# Autodesk Inventor assembly: Ensamblaje4
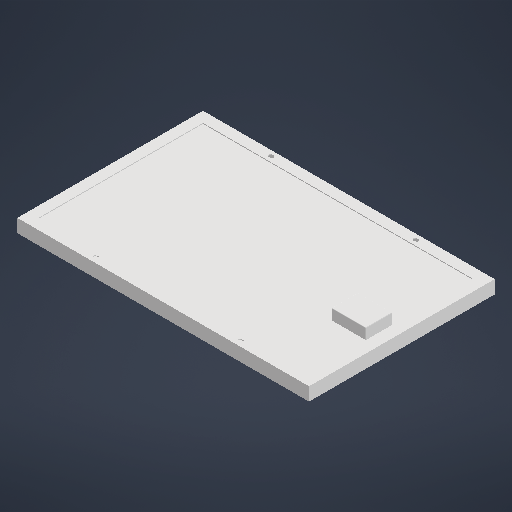
[picture p0: Inventor's stored thumbnail of the model, 512x512]
Saved by Autodesk Inventor 2026.2 (Build 302298000, 298)
## iProperties
Created: 2026-01-05
Part Number: Ensamblaje4
Document SubType Name: Assembly
Designer: vicho
Author: vicho
## Documents named in this file (4)
- C:\Users\vicho\OneDrive\Documentos\PROYECTOS INVENTOR\panel solar\Ensamblaje4.iam
- C:\Users\vicho\OneDrive\Documentos\PROYECTOS INVENTOR\panel solar\marco.ipt
- C:\Users\vicho\OneDrive\Documentos\PROYECTOS INVENTOR\panel solar\panel.ipt
- C:\Users\vicho\OneDrive\Documentos\PROYECTOS INVENTOR\panel solar\componente.ipt
## Components (3 placed, 3 different names)
1. marco:1 — Coincidencia:1, Coincidencia:2, Coincidencia:3, Coincidencia:5, Coincidencia:6
2. panel:1 — Coincidencia:1, Coincidencia:2, Coincidencia:3, Coincidencia:4
3. componente:1 — Coincidencia:4, Coincidencia:5, Coincidencia:6
## Relationships (6: Mate 6)
- Coincidencia:1 [Mate]: marco:1 ↔ panel:1
- Coincidencia:2 [Mate]: marco:1 ↔ panel:1
- Coincidencia:3 [Mate]: marco:1 ↔ panel:1
- Coincidencia:4 [Mate]: panel:1 ↔ componente:1
- Coincidencia:5 [Mate] (40 mm): marco:1 ↔ componente:1
- Coincidencia:6 [Mate] (150 mm): marco:1 ↔ componente:1
